# Autodesk Inventor assembly: Сборка
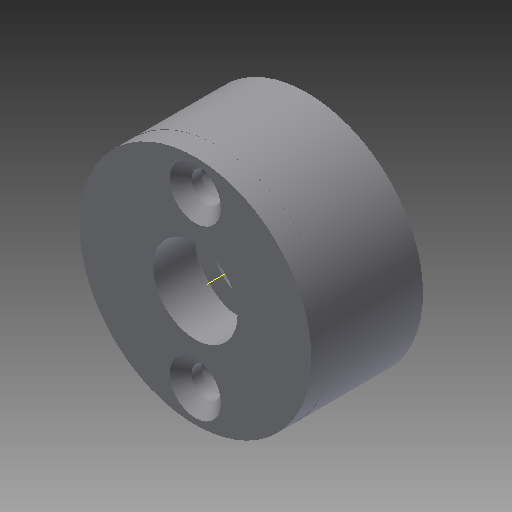
[picture p0: Inventor's stored thumbnail of the model, 512x512]
Saved by Autodesk Inventor 2019 (Build 230136000, 136)
## iProperties
Created: 2019-05-12
Part Number: Сборка
Document SubType Name: Assembly
Mass: 459.912 g
Surface Area: 687.137 cm^2
Volume: 404.227 cm^3
Density: 1.13775 g/cm^3
## Documents named in this file (4)
- C:\Users\STAS-I7\Desktop\Сборка_Стас\Сборка.iam
- C:\Users\STAS-I7\Desktop\Сборка_Стас\Корпус.ipt
- C:\Users\STAS-I7\Desktop\Сборка_Стас\Крышка.ipt
- C:\Users\Juviee\Documents\Inventor\Content Center Files\R2015\ru-RU\GOST 17475-80 (1)\Винт M12-6gx30 ГОСТ 17475-80.ipt
## Components (4 placed, 3 different names)
1. Корпус:1 — Совмещение:1, Совмещение:4
2. Крышка:1 — Совмещение:1, Совмещение:2, Совмещение:3, Совмещение:4
3. Винт ГОСТ 17475-80 M12 x 30:1 — Совмещение:2
4. Винт ГОСТ 17475-80 M12 x 30:2 — Совмещение:3
## Relationships (4: Mate 4)
- Совмещение:1 [Mate]: Корпус:1 ↔ Крышка:1
- Совмещение:2 [Mate]: Крышка:1 ↔ Винт ГОСТ 17475-80 M12 x 30:1
- Совмещение:3 [Mate]: Крышка:1 ↔ Винт ГОСТ 17475-80 M12 x 30:2
- Совмещение:4 [Mate]: Корпус:1 ↔ Крышка:1
